# Autodesk Inventor assembly: EL2-C-100
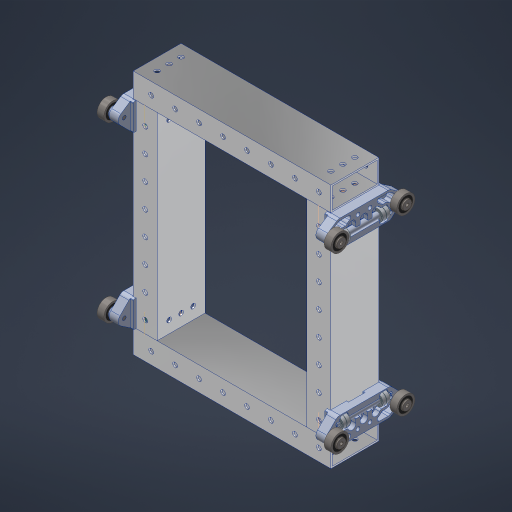
[picture p0: Inventor's stored thumbnail of the model, 512x512]
Saved by Autodesk Inventor 2023.4 (Build 274418000, 418)
## iProperties
Created: 2025-01-11
Part Number: EL2-C-100
Document SubType Name: Assembly
Designer: brand
Author: brand
## Documents named in this file (4)
- C:\Users\brand\OneDrive\Documents\GitHub\robotics 23\2025-ReefScape---CAD\Elevator\EL2\EL2-C-100.iam
- C:\Users\brand\OneDrive\Documents\GitHub\robotics 23\2025-ReefScape---CAD\Elevator\EL2\EL2-C-001.ipt
- C:\Users\brand\OneDrive\Documents\GitHub\robotics 23\2025-ReefScape---CAD\COMMON PARTS\WCP Elevator parts\WCP-0897\WCP-0897.iam
- C:\Users\brand\OneDrive\Documents\GitHub\robotics 23\2025-ReefScape---CAD\Elevator\EL2\EL2-005.ipt
## Components (12 placed, 3 different names)
1. EL2-C-001:1 — Mate:2, Mate:3, Flush:3, Flush:4, Flush:5, Flush:6
2. EL2-C-001:2 — Insert:1, Angle:1, Insert:2, Angle:2, Insert:3, Insert:4, Insert:20, Insert:21, Flush:1, Flush:2, Flush:3, Flush:4
3. EL2-C-001:3 — Insert:8, Angle:3, Insert:9, Insert:10, Angle:4, Insert:22, Insert:23, Flush:5, Flush:6
4. EL2-C-001:4 — Mate:1, Flush:1, Flush:2
5. WCP-0897:1 [sub-assembly] — Insert:9
6. WCP-0897:2 [sub-assembly] — Insert:3, Insert:4
7. EL2-005:1 — Insert:2, Angle:2, Mate:3
8. EL2-005:2 — Insert:8, Angle:3, Mate:2
9. EL2-005:3 — Insert:10, Angle:4
10. EL2-005:4 — Insert:1, Angle:1, Mate:1
11. WCP-0897:3 [sub-assembly] — Insert:22, Insert:23
12. WCP-0897:4 [sub-assembly] — Insert:20, Insert:21
## Relationships (24: Insert 11, Flush 6, Angle 4, Mate 3)
- Insert:1: EL2-C-001:2 ↔ EL2-005:4
- Angle:1 (0 deg): EL2-C-001:2 ↔ EL2-005:4
- Insert:2: EL2-C-001:2 ↔ EL2-005:1
- Angle:2 (0 deg): EL2-C-001:2 ↔ EL2-005:1
- Insert:3: EL2-C-001:2 ↔ WCP-0897:2
- Insert:4: EL2-C-001:2 ↔ WCP-0897:2
- Insert:8: EL2-C-001:3 ↔ EL2-005:2
- Angle:3 (0 deg): EL2-C-001:3 ↔ EL2-005:2
- Insert:9: EL2-C-001:3 ↔ WCP-0897:1
- Insert:10: EL2-C-001:3 ↔ EL2-005:3
- Angle:4 (0 deg): EL2-C-001:3 ↔ EL2-005:3
- Insert:20: EL2-C-001:2 ↔ WCP-0897:4
- Insert:21: EL2-C-001:2 ↔ WCP-0897:4
- Insert:22: EL2-C-001:3 ↔ WCP-0897:3
- Insert:23: EL2-C-001:3 ↔ WCP-0897:3
- Mate:1: EL2-C-001:4 ↔ EL2-005:4
- Flush:1: EL2-C-001:2 ↔ EL2-C-001:4
- Flush:2: EL2-C-001:2 ↔ EL2-C-001:4
- Mate:2: EL2-C-001:1 ↔ EL2-005:2
- Mate:3: EL2-C-001:1 ↔ EL2-005:1
- Flush:3: EL2-C-001:1 ↔ EL2-C-001:2
- Flush:4: EL2-C-001:1 ↔ EL2-C-001:2
- Flush:5: EL2-C-001:1 ↔ EL2-C-001:3
- Flush:6: EL2-C-001:1 ↔ EL2-C-001:3
